# Autodesk Inventor assembly: Base and Exterior Elevator
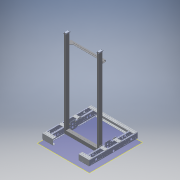
[picture p0: Inventor's stored thumbnail of the model, 180x180]
Saved by Autodesk Inventor 2018 (Build 220112000, 112)
## iProperties
Created: 2015-12-07
Part Number: Base and Exterior Elevator
Description: STEP AP214
Document SubType Name: Assembly
Designer: brooksprench
Sending System: SolidWorks 2014
Preprocessor: SwSTEP 2.0
Title: AM14U3 Square REV1-1.STEP
Revision Number: ANY
## Documents named in this file (7)
- C:\Users\uzair\Documents\School\Clubs\Robotics\CAD for Unity\Base and Exterior Elevator.iam
- C:\Users\uzair\Documents\School\Clubs\Robotics\2018Robot\4992 Robot v0.1\AM14U3 Square Half.iam
- C:\Users\uzair\Documents\School\Clubs\Robotics\2018Robot\4992 Robot v0.1\AM14U3 Square Half Opened.iam
- C:\Users\uzair\Documents\School\Clubs\Robotics\2018Robot\4992 Robot v0.1\4992-2018-Elvator-Exterior Bottom Rail.ipt
- C:\Users\uzair\Documents\School\Clubs\Robotics\2018Robot\4992 Robot v0.1\4992-2018-Elvator-Exterior Side Rail.ipt
- C:\Users\uzair\Documents\School\Clubs\Robotics\2018Robot\4992 Robot v0.1\4992-2018-Elvator-Exterior Side Rail-BentSideRollerPlate.ipt
- C:\Users\uzair\Documents\School\Clubs\Robotics\2018Robot\4992 Robot v0.1\4992-2018-Elvator-Exterior Top Support Member.ipt
## Components (9 placed, 6 different names)
1. AM14U3 Square Half_1 [sub-assembly] — Mate:1, Angle:1, Mate:3, Mate:7
2. AM14U3 Square Half_2 [sub-assembly] — Mate:2, Mate:4, Mate:5, Mate:9, Flush:7
3. 4992-2018-Elvator-Exterior Bottom Rail:1 — Mate:2, Mate:3, Mate:6, Mate:8, Mate:10, Flush:7
4. 4992-2018-Elvator-Exterior Bottom Rail:2 — Mate:4, Mate:5, Mate:6, Flush:1, Flush:2
5. 4992-2018-Elvator-Exterior Side Rail:1 — Mate:7, Mate:8, Flush:1, Mate:12, Flush:3, Flush:4
6. 4992-2018-Elvator-Exterior Side Rail:2 — Mate:9, Mate:10, Flush:2, Mate:11, Flush:5, Flush:6, Mate:27, Flush:19
7. 4992-2018-Elvator-Exterior Side Rail-BentSideRollerPlate:1 — Mate:11, Flush:5, Flush:6
8. 4992-2018-Elvator-Exterior Side Rail-BentSideRollerPlate:2 — Mate:12, Flush:3, Flush:4
9. 4992-2018-Elvator-Exterior Top Support Member:1 — Mate:27, Flush:19
## Relationships (22: Mate 13, Flush 8, Angle 1)
- Mate:1: AM14U3 Square Half_1
- Angle:1 (0 deg): AM14U3 Square Half_1
- Mate:2: AM14U3 Square Half_2 ↔ 4992-2018-Elvator-Exterior Bottom Rail:1
- Mate:3: AM14U3 Square Half_1 ↔ 4992-2018-Elvator-Exterior Bottom Rail:1
- Mate:4: AM14U3 Square Half_2 ↔ 4992-2018-Elvator-Exterior Bottom Rail:2
- Mate:5: AM14U3 Square Half_2 ↔ 4992-2018-Elvator-Exterior Bottom Rail:2
- Mate:6: 4992-2018-Elvator-Exterior Bottom Rail:1 ↔ 4992-2018-Elvator-Exterior Bottom Rail:2
- Mate:7: AM14U3 Square Half_1 ↔ 4992-2018-Elvator-Exterior Side Rail:1
- Mate:8: 4992-2018-Elvator-Exterior Bottom Rail:1 ↔ 4992-2018-Elvator-Exterior Side Rail:1
- Flush:1: 4992-2018-Elvator-Exterior Bottom Rail:2 ↔ 4992-2018-Elvator-Exterior Side Rail:1
- Mate:9: AM14U3 Square Half_2 ↔ 4992-2018-Elvator-Exterior Side Rail:2
- Mate:10: 4992-2018-Elvator-Exterior Bottom Rail:1 ↔ 4992-2018-Elvator-Exterior Side Rail:2
- Flush:2: 4992-2018-Elvator-Exterior Bottom Rail:2 ↔ 4992-2018-Elvator-Exterior Side Rail:2
- Mate:11: 4992-2018-Elvator-Exterior Side Rail:2 ↔ 4992-2018-Elvator-Exterior Side Rail-BentSideRollerPlate:1
- Mate:12: 4992-2018-Elvator-Exterior Side Rail:1 ↔ 4992-2018-Elvator-Exterior Side Rail-BentSideRollerPlate:2
- Flush:3: 4992-2018-Elvator-Exterior Side Rail:1 ↔ 4992-2018-Elvator-Exterior Side Rail-BentSideRollerPlate:2
- Flush:4: 4992-2018-Elvator-Exterior Side Rail:1 ↔ 4992-2018-Elvator-Exterior Side Rail-BentSideRollerPlate:2
- Flush:5: 4992-2018-Elvator-Exterior Side Rail:2 ↔ 4992-2018-Elvator-Exterior Side Rail-BentSideRollerPlate:1
- Flush:6: 4992-2018-Elvator-Exterior Side Rail:2 ↔ 4992-2018-Elvator-Exterior Side Rail-BentSideRollerPlate:1
- Flush:7: AM14U3 Square Half_2 ↔ 4992-2018-Elvator-Exterior Bottom Rail:1
- Mate:27: 4992-2018-Elvator-Exterior Side Rail:2 ↔ 4992-2018-Elvator-Exterior Top Support Member:1
- Flush:19: 4992-2018-Elvator-Exterior Side Rail:2 ↔ 4992-2018-Elvator-Exterior Top Support Member:1
